# Autodesk Inventor assembly: Lower Platform Assembly
Saved by Autodesk Inventor 2014 SP1 (Build 180222100, 222)
## iProperties
Created: 2014-04-09
Part Number: Lower Platform Assembly
Document SubType Name: Assembly
Designer: tom
Author: tom
## Documents named in this file (5)
- C:\Users\tom\Documents\GitHub\Delta_Robots\Delatabot - Small Model\Inventor\Deltabot - Small Model ver12\Lower Platform Assembly.iam
- C:\Users\tom\Documents\GitHub\Delta_Robots\Delatabot - Small Model\Inventor\Deltabot - Small Model ver12\Lower PlatformV.ipt
- C:\Users\tom\Documents\GitHub\Delta_Robots\Delatabot - Small Model\Inventor\Deltabot - Small Model ver12\Lower Arm Bracket.ipt
- C:\Users\tom\Documents\GitHub\Delta_Robots\Delatabot - Small Model\Inventor\Deltabot - Small Model ver12\Linkage Mount.ipt
- C:\Users\tom\Documents\GitHub\Delta_Robots\Delatabot - Small Model\Inventor\Deltabot - Small Model ver12\Bearing.ipt
## Components (13 placed, 4 different names)
1. Lower PlatformV:1
2. Lower Arm Bracket:1
3. Linkage Mount:1
4. Bearing:1
5. Bearing:2
6. Lower Arm Bracket:2
7. Linkage Mount:2
8. Bearing:3
9. Bearing:5
10. Lower Arm Bracket:3
11. Linkage Mount:3
12. Bearing:4
13. Bearing:6
## Component patterns: (3 elements, first: Lower Arm Bracket:1 + Linkage Mount:1 + Bearing:1 + Bearing:2)
## Relationships (7: Mate 5, RevoluteJoint 2)
- [Mate]: Lower PlatformV:1 ↔ Lower Arm Bracket:1
- [Mate]: Lower PlatformV:1 ↔ Lower Arm Bracket:1
- [Mate]: Lower PlatformV:1 ↔ Lower Arm Bracket:1
- [Mate]: Lower Arm Bracket:1 ↔ Linkage Mount:1
- [Mate] (6.67 mm): Lower Arm Bracket:1 ↔ Linkage Mount:1
- [RevoluteJoint]: Linkage Mount:1 ↔ Bearing:1
- [RevoluteJoint]: Linkage Mount:1 ↔ Bearing:2
